# Autodesk Inventor assembly: Lap rap truc Y
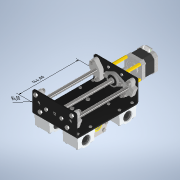
[picture p0: Inventor's stored thumbnail of the model, 180x180]
Saved by Autodesk Inventor 2021 (Build 250183000, 183)
## iProperties
Created: 2021-05-26
Part Number: Lap rap truc Y
Document SubType Name: Assembly
Designer: admin
Author: admin
## Documents named in this file (21)
- C:\Users\79449\Documents\CNC_DISENO_DE MAQUINAS\Piezas-Ensambles_Inventor\Segunda_presentación\Lap rap truc Y.iam
- C:\Users\79449\Documents\CNC_DISENO_DE MAQUINAS\Piezas-Ensambles_Inventor\Segunda_presentación\De  truc Y.ipt
- C:\Users\79449\Documents\CNC_DISENO_DE MAQUINAS\Piezas-Ensambles_Inventor\Segunda_presentación\Kep Truc KLF-08.ipt
- C:\Users\79449\Documents\CNC_DISENO_DE MAQUINAS\Piezas-Ensambles_Inventor\Segunda_presentación\Nema17\Assembly1.iam
- C:\Users\79449\Documents\CNC_DISENO_DE MAQUINAS\Piezas-Ensambles_Inventor\Segunda_presentación\Tru dong 40mm.ipt
- C:\Users\79449\Documents\CNC_DISENO_DE MAQUINAS\Piezas-Ensambles_Inventor\Segunda_presentación\SC12uu\PILLOW 12MM FINAL.iam
- C:\Users\79449\Documents\CNC_DISENO_DE MAQUINAS\Piezas-Ensambles_Inventor\Segunda_presentación\Flexible Coupling 8,8.ipt
- C:\Users\79449\Documents\CNC_DISENO_DE MAQUINAS\Piezas-Ensambles_Inventor\Segunda_presentación\Vitme T8 dai 200mm.ipt
- C:\Users\79449\Documents\CNC_DISENO_DE MAQUINAS\Piezas-Ensambles_Inventor\Segunda_presentación\SHF08.ipt
- C:\Users\79449\Documents\CNC_DISENO_DE MAQUINAS\Piezas-Ensambles_Inventor\Segunda_presentación\EjeBase.ipt
- C:\Users\79449\Documents\CNC_DISENO_DE MAQUINAS\Piezas-Ensambles_Inventor\Segunda_presentación\ball nut housing bracket holder.ipt
- C:\Users\79449\Documents\CNC_DISENO_DE MAQUINAS\Piezas-Ensambles_Inventor\Segunda_presentación\SFU-1605.ipt
- C:\Users\79449\Documents\Inventor\Content Center Files\R2021\es-ES\AS 1110\AS 1110 - M5 x 20.ipt
- C:\Users\79449\Documents\Inventor\Content Center Files\R2021\es-ES\AS 1110\AS 1110 - M2,5 x 6.ipt
- C:\Users\79449\Documents\Inventor\Content Center Files\R2021\es-ES\AS 1110\AS 1110 - M4 x 12.ipt
- C:\Users\79449\Documents\Inventor\Content Center Files\R2021\es-ES\AS 1110\AS 1110 - M3 x 30.ipt
- C:\Users\79449\Documents\Inventor\Content Center Files\R2021\es-ES\AS 1110\AS 1110 - M4 x 8.ipt
- C:\Users\79449\Documents\Inventor\Content Center Files\R2021\es-ES\AS 1110\AS 1110 - M4 x 20.ipt
- C:\Users\79449\Documents\Inventor\Content Center Files\R2021\es-ES\ANSI B18.2.4.2M\ANSI B18.2.4.2M - M5x0,8 - 8.ipt
- C:\Users\79449\Documents\Inventor\Content Center Files\R2021\es-ES\ANSI B18.2.4.2M\ANSI B18.2.4.2M - M4x0,7 - 7.ipt
- C:\Users\79449\Documents\Inventor\Content Center Files\R2021\es-ES\ANSI B18.2.4.2M\ANSI B18.2.4.2M - M3x0,5 - 5,5.ipt
## Components (92 placed, 20 different names)
1. De  truc Y:1 — Mate:4, Mate:5, Mate:6, Mate:13, Mate:15, Mate:16, Mate:21, Mate:22, Mate:23, Mate:24, Mate:25, Mate:26, Mate:27, Mate:28, Mate:37, Mate:38, Mate:39, Mate:48, Mate:53, Mate:54, Mate:57, Mate:58, Mate:59, Mate:60, Mate:63, Mate:64, Mate:65, Ángulo:1, Coincidencia:70, Coincidencia:71, Coincidencia:73, Coincidencia:74, Coincidencia:75, Coincidencia:76, Coincidencia:77, Coincidencia:78, Coincidencia:79, Coincidencia:80, Coincidencia:81, Coincidencia:82, Coincidencia:83, Coincidencia:85, Coincidencia:86, Coincidencia:87, Coincidencia:91, Coincidencia:93, Coincidencia:95, Coincidencia:97, Coincidencia:99, Coincidencia:101, Coincidencia:103, Coincidencia:105, Coincidencia:107, Coincidencia:111, Coincidencia:113, Coincidencia:115, Coincidencia:117, Coincidencia:119, Coincidencia:121, Coincidencia:123, Coincidencia:125, Coincidencia:127, Coincidencia:129, Coincidencia:131, Coincidencia:133, Coincidencia:135, Coincidencia:137, Coincidencia:139, Coincidencia:141, Coincidencia:143, Coincidencia:145, Coincidencia:147, Coincidencia:149, Coincidencia:151, Coincidencia:153, Coincidencia:155, Coincidencia:157, Coincidencia:219, Coincidencia:221, Coincidencia:223, Coincidencia:225
2. Assembly1:1 [sub-assembly] — Coincidencia:69, Ángulo:1
3. Kep Truc KLF-08:2 — Mate:4, Mate:5, Mate:6, Coincidencia:118, Coincidencia:120, Coincidencia:187, Coincidencia:189
4. Kep Truc KLF-08:3 — Mate:13, Mate:15, Mate:16, Mate:19, Coincidencia:122, Coincidencia:124, Coincidencia:191, Coincidencia:193
5. Vitme T8 dai 200mm:1 — Mate:19, Coincidencia:90
6. Tru dong 40mm:1 — Mate:22, Mate:26, Coincidencia:110
7. Tru dong 40mm:2 — Mate:21, Mate:25, Coincidencia:116
8. Tru dong 40mm:3 — Mate:24, Mate:28, Coincidencia:114
9. Tru dong 40mm:4 — Mate:23, Mate:27, Coincidencia:69, Coincidencia:112
10. PILLOW 12MM FINAL:5 [sub-assembly] — Mate:37, Mate:38, Mate:39, Coincidencia:77, Coincidencia:78, Coincidencia:126, Coincidencia:128, Coincidencia:130, Coincidencia:132, Coincidencia:203, Coincidencia:205, Coincidencia:207, Coincidencia:209
11. PILLOW 12MM FINAL:6 [sub-assembly] — Mate:48, Coincidencia:79, Coincidencia:80, Coincidencia:218, Coincidencia:220, Coincidencia:222, Coincidencia:224, Coincidencia:227, Coincidencia:229, Coincidencia:231, Coincidencia:233
12. PILLOW 12MM FINAL:7 [sub-assembly] — Flush:1, Flush:2, Mate:53, Coincidencia:75, Coincidencia:76, Coincidencia:83, Coincidencia:134, Coincidencia:136, Coincidencia:138, Coincidencia:140, Coincidencia:195, Coincidencia:197, Coincidencia:199, Coincidencia:201
13. PILLOW 12MM FINAL:8 [sub-assembly] — Flush:1, Flush:2, Coincidencia:81, Coincidencia:82, Coincidencia:142, Coincidencia:144, Coincidencia:146, Coincidencia:148, Coincidencia:211, Coincidencia:213, Coincidencia:215, Coincidencia:217
14. SHF08:1 — Mate:54, Coincidencia:72, Coincidencia:100, Coincidencia:102, Coincidencia:171, Coincidencia:173
15. SHF08:2 — Mate:60, Coincidencia:74, Coincidencia:92, Coincidencia:94, Coincidencia:183, Coincidencia:185
16. SHF08:3 — Mate:63, Mate:64, Mate:65, Coincidencia:96, Coincidencia:98, Coincidencia:179, Coincidencia:181
17. SHF08:4 — Mate:57, Mate:58, Mate:59, Coincidencia:104, Coincidencia:106, Coincidencia:175, Coincidencia:177
18. EjeBase:1 — Coincidencia:70, Coincidencia:71
19. EjeBase:2 — Coincidencia:72, Coincidencia:73
20. ball nut housing bracket holder:1 — Coincidencia:85, Coincidencia:86, Coincidencia:87, Coincidencia:88, Ángulo:2, Coincidencia:89, Coincidencia:150, Coincidencia:152, Coincidencia:154, Coincidencia:156, Coincidencia:158, Coincidencia:160, Coincidencia:162, Coincidencia:164, Coincidencia:166, Coincidencia:168
21. SFU-1605:1 — Coincidencia:88, Ángulo:2, Coincidencia:89, Coincidencia:159, Coincidencia:161, Coincidencia:163, Coincidencia:165, Coincidencia:167, Coincidencia:169
22. Flexible Coupling 8,8:1 — Coincidencia:90, Coincidencia:91
23. AS 1110 - Métrico M5 x 20:1 — Coincidencia:92, Coincidencia:93, Coincidencia:182
24. AS 1110 - Métrico M5 x 20:2 — Coincidencia:94, Coincidencia:95, Coincidencia:184
25. AS 1110 - Métrico M5 x 20:3 — Coincidencia:96, Coincidencia:97, Coincidencia:178
26. AS 1110 - Métrico M5 x 20:4 — Coincidencia:98, Coincidencia:99, Coincidencia:180
27. AS 1110 - Métrico M5 x 20:5 — Coincidencia:100, Coincidencia:101, Coincidencia:170
28. AS 1110 - Métrico M5 x 20:6 — Coincidencia:102, Coincidencia:103, Coincidencia:172
29. AS 1110 - Métrico M5 x 20:7 — Coincidencia:104, Coincidencia:105, Coincidencia:174
30. AS 1110 - Métrico M5 x 20:8 — Coincidencia:106, Coincidencia:107, Coincidencia:176
31. AS 1110 - Métrico M2,5 x 6:2 — Coincidencia:110, Coincidencia:111
32. AS 1110 - Métrico M2,5 x 6:3 — Coincidencia:112, Coincidencia:113
33. AS 1110 - Métrico M2,5 x 6:4 — Coincidencia:114, Coincidencia:115
34. AS 1110 - Métrico M2,5 x 6:5 — Coincidencia:116, Coincidencia:117
35. AS 1110 - Métrico M4 x 12:1 — Coincidencia:118, Coincidencia:119, Coincidencia:188
36. AS 1110 - Métrico M4 x 12:2 — Coincidencia:120, Coincidencia:121, Coincidencia:186
37. AS 1110 - Métrico M4 x 12:3 — Coincidencia:122, Coincidencia:123, Coincidencia:192
38. AS 1110 - Métrico M4 x 12:4 — Coincidencia:124, Coincidencia:125, Coincidencia:190
39. AS 1110 - Métrico M3 x 30:1 — Coincidencia:126, Coincidencia:127, Coincidencia:206
40. AS 1110 - Métrico M3 x 30:2 — Coincidencia:128, Coincidencia:129, Coincidencia:208
41. AS 1110 - Métrico M3 x 30:3 — Coincidencia:130, Coincidencia:131, Coincidencia:204
42. AS 1110 - Métrico M3 x 30:4 — Coincidencia:132, Coincidencia:133, Coincidencia:202
43. AS 1110 - Métrico M3 x 30:5 — Coincidencia:134, Coincidencia:135, Coincidencia:194
44. AS 1110 - Métrico M3 x 30:6 — Coincidencia:136, Coincidencia:137, Coincidencia:196
45. AS 1110 - Métrico M3 x 30:7 — Coincidencia:138, Coincidencia:139, Coincidencia:200
46. AS 1110 - Métrico M3 x 30:8 — Coincidencia:140, Coincidencia:141, Coincidencia:198
47. AS 1110 - Métrico M3 x 30:9 — Coincidencia:142, Coincidencia:143, Coincidencia:216
48. AS 1110 - Métrico M3 x 30:10 — Coincidencia:144, Coincidencia:145, Coincidencia:210
49. AS 1110 - Métrico M3 x 30:11 — Coincidencia:146, Coincidencia:147, Coincidencia:214
50. AS 1110 - Métrico M3 x 30:12 — Coincidencia:148, Coincidencia:149, Coincidencia:212
51. AS 1110 - Métrico M4 x 8:1 — Coincidencia:150, Coincidencia:151
52. AS 1110 - Métrico M4 x 8:2 — Coincidencia:152, Coincidencia:153
53. AS 1110 - Métrico M4 x 8:3 — Coincidencia:154, Coincidencia:155
54. AS 1110 - Métrico M4 x 8:4 — Coincidencia:156, Coincidencia:157
55. AS 1110 - Métrico M4 x 20:1 — Coincidencia:158, Coincidencia:159
56. AS 1110 - Métrico M4 x 20:2 — Coincidencia:160, Coincidencia:161
57. AS 1110 - Métrico M4 x 20:3 — Coincidencia:162, Coincidencia:163
58. AS 1110 - Métrico M4 x 20:4 — Coincidencia:164, Coincidencia:165
59. AS 1110 - Métrico M4 x 20:5 — Coincidencia:166, Coincidencia:167
60. AS 1110 - Métrico M4 x 20:6 — Coincidencia:168, Coincidencia:169
61. ANSI B18.2.4.2M M5x0,8:1 — Coincidencia:170, Coincidencia:171
62. ANSI B18.2.4.2M M5x0,8:2 — Coincidencia:172, Coincidencia:173
63. ANSI B18.2.4.2M M5x0,8:3 — Coincidencia:174, Coincidencia:175
64. ANSI B18.2.4.2M M5x0,8:4 — Coincidencia:176, Coincidencia:177
65. ANSI B18.2.4.2M M5x0,8:5 — Coincidencia:178, Coincidencia:179
66. ANSI B18.2.4.2M M5x0,8:6 — Coincidencia:180, Coincidencia:181
67. ANSI B18.2.4.2M M5x0,8:7 — Coincidencia:182, Coincidencia:183
68. ANSI B18.2.4.2M M5x0,8:8 — Coincidencia:184, Coincidencia:185
69. ANSI B18.2.4.2M M4x0,7:1 — Coincidencia:186, Coincidencia:187
70. ANSI B18.2.4.2M M4x0,7:2 — Coincidencia:188, Coincidencia:189
71. ANSI B18.2.4.2M M4x0,7:3 — Coincidencia:190, Coincidencia:191
72. ANSI B18.2.4.2M M4x0,7:4 — Coincidencia:192, Coincidencia:193
73. ANSI B18.2.4.2M M3x0,5:1 — Coincidencia:194, Coincidencia:195
74. ANSI B18.2.4.2M M3x0,5:2 — Coincidencia:196, Coincidencia:197
75. ANSI B18.2.4.2M M3x0,5:3 — Coincidencia:198, Coincidencia:199
76. ANSI B18.2.4.2M M3x0,5:4 — Coincidencia:200, Coincidencia:201
77. ANSI B18.2.4.2M M3x0,5:5 — Coincidencia:202, Coincidencia:203
78. ANSI B18.2.4.2M M3x0,5:6 — Coincidencia:204, Coincidencia:205
79. ANSI B18.2.4.2M M3x0,5:7 — Coincidencia:206, Coincidencia:207
80. ANSI B18.2.4.2M M3x0,5:8 — Coincidencia:208, Coincidencia:209
81. ANSI B18.2.4.2M M3x0,5:9 — Coincidencia:210, Coincidencia:211
82. ANSI B18.2.4.2M M3x0,5:10 — Coincidencia:212, Coincidencia:213
83. ANSI B18.2.4.2M M3x0,5:11 — Coincidencia:214, Coincidencia:215
84. ANSI B18.2.4.2M M3x0,5:12 — Coincidencia:216, Coincidencia:217
85. AS 1110 - Métrico M3 x 30:13 — Coincidencia:218, Coincidencia:219, Coincidencia:232
86. AS 1110 - Métrico M3 x 30:14 — Coincidencia:220, Coincidencia:221, Coincidencia:230
87. AS 1110 - Métrico M3 x 30:15 — Coincidencia:222, Coincidencia:223, Coincidencia:226
88. AS 1110 - Métrico M3 x 30:16 — Coincidencia:224, Coincidencia:225, Coincidencia:228
89. ANSI B18.2.4.2M M3x0,5:13 — Coincidencia:226, Coincidencia:227
90. ANSI B18.2.4.2M M3x0,5:14 — Coincidencia:228, Coincidencia:229
91. ANSI B18.2.4.2M M3x0,5:15 — Coincidencia:230, Coincidencia:231
92. ANSI B18.2.4.2M M3x0,5:16 — Coincidencia:232, Coincidencia:233
## Relationships (194: Mate 190, Flush 2, Angle 2)
- Mate:4: De  truc Y:1 ↔ Kep Truc KLF-08:2
- Mate:5: De  truc Y:1 ↔ Kep Truc KLF-08:2
- Mate:6: De  truc Y:1 ↔ Kep Truc KLF-08:2
- Mate:13: De  truc Y:1 ↔ Kep Truc KLF-08:3
- Mate:15: De  truc Y:1 ↔ Kep Truc KLF-08:3
- Mate:16: De  truc Y:1 ↔ Kep Truc KLF-08:3
- Mate:19: Kep Truc KLF-08:3 ↔ Vitme T8 dai 200mm:1
- Mate:21: De  truc Y:1 ↔ Tru dong 40mm:2
- Mate:22: De  truc Y:1 ↔ Tru dong 40mm:1
- Mate:23: De  truc Y:1 ↔ Tru dong 40mm:4
- Mate:24: De  truc Y:1 ↔ Tru dong 40mm:3
- Mate:25: De  truc Y:1 ↔ Tru dong 40mm:2
- Mate:26: De  truc Y:1 ↔ Tru dong 40mm:1
- Mate:27: De  truc Y:1 ↔ Tru dong 40mm:4
- Mate:28: De  truc Y:1 ↔ Tru dong 40mm:3
- Mate:37: De  truc Y:1 ↔ PILLOW 12MM FINAL:5
- Mate:38: De  truc Y:1 ↔ PILLOW 12MM FINAL:5
- Mate:39: De  truc Y:1 ↔ PILLOW 12MM FINAL:5
- Mate:48: De  truc Y:1 ↔ PILLOW 12MM FINAL:6
- Flush:1: PILLOW 12MM FINAL:7 ↔ PILLOW 12MM FINAL:8
- Flush:2: PILLOW 12MM FINAL:7 ↔ PILLOW 12MM FINAL:8
- Mate:53: De  truc Y:1 ↔ PILLOW 12MM FINAL:7
- Mate:54: De  truc Y:1 ↔ SHF08:1
- Mate:57: De  truc Y:1 ↔ SHF08:4
- Mate:58: De  truc Y:1 ↔ SHF08:4
- Mate:59: De  truc Y:1 ↔ SHF08:4
- Mate:60: De  truc Y:1 ↔ SHF08:2
- Mate:63: De  truc Y:1 ↔ SHF08:3
- Mate:64: De  truc Y:1 ↔ SHF08:3
- Mate:65: De  truc Y:1 ↔ SHF08:3
- Coincidencia:69 [Mate]: Assembly1:1 ↔ Tru dong 40mm:4
- Ángulo:1 [Angle] (0 deg): De  truc Y:1 ↔ Assembly1:1
- Coincidencia:70 [Mate]: De  truc Y:1 ↔ EjeBase:1
- Coincidencia:71 [Mate]: De  truc Y:1 ↔ EjeBase:1
- Coincidencia:72 [Mate]: SHF08:1 ↔ EjeBase:2
- Coincidencia:73 [Mate]: De  truc Y:1 ↔ EjeBase:2
- Coincidencia:74 [Mate]: De  truc Y:1 ↔ SHF08:2
- Coincidencia:75 [Mate]: De  truc Y:1 ↔ PILLOW 12MM FINAL:7
- Coincidencia:76 [Mate]: De  truc Y:1 ↔ PILLOW 12MM FINAL:7
- Coincidencia:77 [Mate]: De  truc Y:1 ↔ PILLOW 12MM FINAL:5
- Coincidencia:78 [Mate]: De  truc Y:1 ↔ PILLOW 12MM FINAL:5
- Coincidencia:79 [Mate]: De  truc Y:1 ↔ PILLOW 12MM FINAL:6
- Coincidencia:80 [Mate]: De  truc Y:1 ↔ PILLOW 12MM FINAL:6
- Coincidencia:81 [Mate]: De  truc Y:1 ↔ PILLOW 12MM FINAL:8
- Coincidencia:82 [Mate]: De  truc Y:1 ↔ PILLOW 12MM FINAL:8
- Coincidencia:83 [Mate]: De  truc Y:1 ↔ PILLOW 12MM FINAL:7
- Coincidencia:85 [Mate]: De  truc Y:1 ↔ ball nut housing bracket holder:1
- Coincidencia:86 [Mate]: De  truc Y:1 ↔ ball nut housing bracket holder:1
- Coincidencia:87 [Mate]: De  truc Y:1 ↔ ball nut housing bracket holder:1
- Coincidencia:88 [Mate]: ball nut housing bracket holder:1 ↔ SFU-1605:1
- Ángulo:2 [Angle] (0 deg): ball nut housing bracket holder:1 ↔ SFU-1605:1
- Coincidencia:89 [Mate]: ball nut housing bracket holder:1 ↔ SFU-1605:1
- Coincidencia:90 [Mate]: Vitme T8 dai 200mm:1 ↔ Flexible Coupling 8,8:1
- Coincidencia:91 [Mate]: De  truc Y:1 ↔ Flexible Coupling 8,8:1
- Coincidencia:92 [Mate]: SHF08:2 ↔ AS 1110 - Métrico M5 x 20:1
- Coincidencia:93 [Mate]: De  truc Y:1 ↔ AS 1110 - Métrico M5 x 20:1
- Coincidencia:94 [Mate]: SHF08:2 ↔ AS 1110 - Métrico M5 x 20:2
- Coincidencia:95 [Mate]: De  truc Y:1 ↔ AS 1110 - Métrico M5 x 20:2
- Coincidencia:96 [Mate]: SHF08:3 ↔ AS 1110 - Métrico M5 x 20:3
- Coincidencia:97 [Mate]: De  truc Y:1 ↔ AS 1110 - Métrico M5 x 20:3
- Coincidencia:98 [Mate]: SHF08:3 ↔ AS 1110 - Métrico M5 x 20:4
- Coincidencia:99 [Mate]: De  truc Y:1 ↔ AS 1110 - Métrico M5 x 20:4
- Coincidencia:100 [Mate]: SHF08:1 ↔ AS 1110 - Métrico M5 x 20:5
- Coincidencia:101 [Mate]: De  truc Y:1 ↔ AS 1110 - Métrico M5 x 20:5
- Coincidencia:102 [Mate]: SHF08:1 ↔ AS 1110 - Métrico M5 x 20:6
- Coincidencia:103 [Mate]: De  truc Y:1 ↔ AS 1110 - Métrico M5 x 20:6
- Coincidencia:104 [Mate]: SHF08:4 ↔ AS 1110 - Métrico M5 x 20:7
- Coincidencia:105 [Mate]: De  truc Y:1 ↔ AS 1110 - Métrico M5 x 20:7
- Coincidencia:106 [Mate]: SHF08:4 ↔ AS 1110 - Métrico M5 x 20:8
- Coincidencia:107 [Mate]: De  truc Y:1 ↔ AS 1110 - Métrico M5 x 20:8
- Coincidencia:110 [Mate]: Tru dong 40mm:1 ↔ AS 1110 - Métrico M2,5 x 6:2
- Coincidencia:111 [Mate]: De  truc Y:1 ↔ AS 1110 - Métrico M2,5 x 6:2
- Coincidencia:112 [Mate]: Tru dong 40mm:4 ↔ AS 1110 - Métrico M2,5 x 6:3
- Coincidencia:113 [Mate]: De  truc Y:1 ↔ AS 1110 - Métrico M2,5 x 6:3
- Coincidencia:114 [Mate]: Tru dong 40mm:3 ↔ AS 1110 - Métrico M2,5 x 6:4
- Coincidencia:115 [Mate]: De  truc Y:1 ↔ AS 1110 - Métrico M2,5 x 6:4
- Coincidencia:116 [Mate]: Tru dong 40mm:2 ↔ AS 1110 - Métrico M2,5 x 6:5
- Coincidencia:117 [Mate]: De  truc Y:1 ↔ AS 1110 - Métrico M2,5 x 6:5
- Coincidencia:118 [Mate]: Kep Truc KLF-08:2 ↔ AS 1110 - Métrico M4 x 12:1
- Coincidencia:119 [Mate]: De  truc Y:1 ↔ AS 1110 - Métrico M4 x 12:1
- Coincidencia:120 [Mate]: Kep Truc KLF-08:2 ↔ AS 1110 - Métrico M4 x 12:2
- Coincidencia:121 [Mate]: De  truc Y:1 ↔ AS 1110 - Métrico M4 x 12:2
- Coincidencia:122 [Mate]: Kep Truc KLF-08:3 ↔ AS 1110 - Métrico M4 x 12:3
- Coincidencia:123 [Mate]: De  truc Y:1 ↔ AS 1110 - Métrico M4 x 12:3
- Coincidencia:124 [Mate]: Kep Truc KLF-08:3 ↔ AS 1110 - Métrico M4 x 12:4
- Coincidencia:125 [Mate]: De  truc Y:1 ↔ AS 1110 - Métrico M4 x 12:4
- Coincidencia:126 [Mate]: PILLOW 12MM FINAL:5 ↔ AS 1110 - Métrico M3 x 30:1
- Coincidencia:127 [Mate]: De  truc Y:1 ↔ AS 1110 - Métrico M3 x 30:1
- Coincidencia:128 [Mate]: PILLOW 12MM FINAL:5 ↔ AS 1110 - Métrico M3 x 30:2
- Coincidencia:129 [Mate]: De  truc Y:1 ↔ AS 1110 - Métrico M3 x 30:2
- Coincidencia:130 [Mate]: PILLOW 12MM FINAL:5 ↔ AS 1110 - Métrico M3 x 30:3
- Coincidencia:131 [Mate]: De  truc Y:1 ↔ AS 1110 - Métrico M3 x 30:3
- Coincidencia:132 [Mate]: PILLOW 12MM FINAL:5 ↔ AS 1110 - Métrico M3 x 30:4
- Coincidencia:133 [Mate]: De  truc Y:1 ↔ AS 1110 - Métrico M3 x 30:4
- Coincidencia:134 [Mate]: PILLOW 12MM FINAL:7 ↔ AS 1110 - Métrico M3 x 30:5
- Coincidencia:135 [Mate]: De  truc Y:1 ↔ AS 1110 - Métrico M3 x 30:5
- Coincidencia:136 [Mate]: PILLOW 12MM FINAL:7 ↔ AS 1110 - Métrico M3 x 30:6
- Coincidencia:137 [Mate]: De  truc Y:1 ↔ AS 1110 - Métrico M3 x 30:6
- Coincidencia:138 [Mate]: PILLOW 12MM FINAL:7 ↔ AS 1110 - Métrico M3 x 30:7
- Coincidencia:139 [Mate]: De  truc Y:1 ↔ AS 1110 - Métrico M3 x 30:7
- Coincidencia:140 [Mate]: PILLOW 12MM FINAL:7 ↔ AS 1110 - Métrico M3 x 30:8
- Coincidencia:141 [Mate]: De  truc Y:1 ↔ AS 1110 - Métrico M3 x 30:8
- Coincidencia:142 [Mate]: PILLOW 12MM FINAL:8 ↔ AS 1110 - Métrico M3 x 30:9
- Coincidencia:143 [Mate]: De  truc Y:1 ↔ AS 1110 - Métrico M3 x 30:9
- Coincidencia:144 [Mate]: PILLOW 12MM FINAL:8 ↔ AS 1110 - Métrico M3 x 30:10
- Coincidencia:145 [Mate]: De  truc Y:1 ↔ AS 1110 - Métrico M3 x 30:10
- Coincidencia:146 [Mate]: PILLOW 12MM FINAL:8 ↔ AS 1110 - Métrico M3 x 30:11
- Coincidencia:147 [Mate]: De  truc Y:1 ↔ AS 1110 - Métrico M3 x 30:11
- Coincidencia:148 [Mate]: PILLOW 12MM FINAL:8 ↔ AS 1110 - Métrico M3 x 30:12
- Coincidencia:149 [Mate]: De  truc Y:1 ↔ AS 1110 - Métrico M3 x 30:12
- Coincidencia:150 [Mate]: ball nut housing bracket holder:1 ↔ AS 1110 - Métrico M4 x 8:1
- Coincidencia:151 [Mate]: De  truc Y:1 ↔ AS 1110 - Métrico M4 x 8:1
- Coincidencia:152 [Mate]: ball nut housing bracket holder:1 ↔ AS 1110 - Métrico M4 x 8:2
- Coincidencia:153 [Mate]: De  truc Y:1 ↔ AS 1110 - Métrico M4 x 8:2
- Coincidencia:154 [Mate]: ball nut housing bracket holder:1 ↔ AS 1110 - Métrico M4 x 8:3
- Coincidencia:155 [Mate]: De  truc Y:1 ↔ AS 1110 - Métrico M4 x 8:3
- Coincidencia:156 [Mate]: ball nut housing bracket holder:1 ↔ AS 1110 - Métrico M4 x 8:4
- Coincidencia:157 [Mate]: De  truc Y:1 ↔ AS 1110 - Métrico M4 x 8:4
- Coincidencia:158 [Mate]: ball nut housing bracket holder:1 ↔ AS 1110 - Métrico M4 x 20:1
- Coincidencia:159 [Mate]: SFU-1605:1 ↔ AS 1110 - Métrico M4 x 20:1
- Coincidencia:160 [Mate]: ball nut housing bracket holder:1 ↔ AS 1110 - Métrico M4 x 20:2
- Coincidencia:161 [Mate]: SFU-1605:1 ↔ AS 1110 - Métrico M4 x 20:2
- Coincidencia:162 [Mate]: ball nut housing bracket holder:1 ↔ AS 1110 - Métrico M4 x 20:3
- Coincidencia:163 [Mate]: SFU-1605:1 ↔ AS 1110 - Métrico M4 x 20:3
- Coincidencia:164 [Mate]: ball nut housing bracket holder:1 ↔ AS 1110 - Métrico M4 x 20:4
- Coincidencia:165 [Mate]: SFU-1605:1 ↔ AS 1110 - Métrico M4 x 20:4
- Coincidencia:166 [Mate]: ball nut housing bracket holder:1 ↔ AS 1110 - Métrico M4 x 20:5
- Coincidencia:167 [Mate]: SFU-1605:1 ↔ AS 1110 - Métrico M4 x 20:5
- Coincidencia:168 [Mate]: ball nut housing bracket holder:1 ↔ AS 1110 - Métrico M4 x 20:6
- Coincidencia:169 [Mate]: SFU-1605:1 ↔ AS 1110 - Métrico M4 x 20:6
- Coincidencia:170 [Mate]: AS 1110 - Métrico M5 x 20:5 ↔ ANSI B18.2.4.2M M5x0,8:1
- Coincidencia:171 [Mate]: SHF08:1 ↔ ANSI B18.2.4.2M M5x0,8:1
- Coincidencia:172 [Mate]: AS 1110 - Métrico M5 x 20:6 ↔ ANSI B18.2.4.2M M5x0,8:2
- Coincidencia:173 [Mate]: SHF08:1 ↔ ANSI B18.2.4.2M M5x0,8:2
- Coincidencia:174 [Mate]: AS 1110 - Métrico M5 x 20:7 ↔ ANSI B18.2.4.2M M5x0,8:3
- Coincidencia:175 [Mate]: SHF08:4 ↔ ANSI B18.2.4.2M M5x0,8:3
- Coincidencia:176 [Mate]: AS 1110 - Métrico M5 x 20:8 ↔ ANSI B18.2.4.2M M5x0,8:4
- Coincidencia:177 [Mate]: SHF08:4 ↔ ANSI B18.2.4.2M M5x0,8:4
- Coincidencia:178 [Mate]: AS 1110 - Métrico M5 x 20:3 ↔ ANSI B18.2.4.2M M5x0,8:5
- Coincidencia:179 [Mate]: SHF08:3 ↔ ANSI B18.2.4.2M M5x0,8:5
- Coincidencia:180 [Mate]: AS 1110 - Métrico M5 x 20:4 ↔ ANSI B18.2.4.2M M5x0,8:6
- Coincidencia:181 [Mate]: SHF08:3 ↔ ANSI B18.2.4.2M M5x0,8:6
- Coincidencia:182 [Mate]: AS 1110 - Métrico M5 x 20:1 ↔ ANSI B18.2.4.2M M5x0,8:7
- Coincidencia:183 [Mate]: SHF08:2 ↔ ANSI B18.2.4.2M M5x0,8:7
- Coincidencia:184 [Mate]: AS 1110 - Métrico M5 x 20:2 ↔ ANSI B18.2.4.2M M5x0,8:8
- Coincidencia:185 [Mate]: SHF08:2 ↔ ANSI B18.2.4.2M M5x0,8:8
- Coincidencia:186 [Mate]: AS 1110 - Métrico M4 x 12:2 ↔ ANSI B18.2.4.2M M4x0,7:1
- Coincidencia:187 [Mate]: Kep Truc KLF-08:2 ↔ ANSI B18.2.4.2M M4x0,7:1
- Coincidencia:188 [Mate]: AS 1110 - Métrico M4 x 12:1 ↔ ANSI B18.2.4.2M M4x0,7:2
- Coincidencia:189 [Mate]: Kep Truc KLF-08:2 ↔ ANSI B18.2.4.2M M4x0,7:2
- Coincidencia:190 [Mate]: AS 1110 - Métrico M4 x 12:4 ↔ ANSI B18.2.4.2M M4x0,7:3
- Coincidencia:191 [Mate]: Kep Truc KLF-08:3 ↔ ANSI B18.2.4.2M M4x0,7:3
- Coincidencia:192 [Mate]: AS 1110 - Métrico M4 x 12:3 ↔ ANSI B18.2.4.2M M4x0,7:4
- Coincidencia:193 [Mate]: Kep Truc KLF-08:3 ↔ ANSI B18.2.4.2M M4x0,7:4
- Coincidencia:194 [Mate]: AS 1110 - Métrico M3 x 30:5 ↔ ANSI B18.2.4.2M M3x0,5:1
- Coincidencia:195 [Mate]: PILLOW 12MM FINAL:7 ↔ ANSI B18.2.4.2M M3x0,5:1
- Coincidencia:196 [Mate]: AS 1110 - Métrico M3 x 30:6 ↔ ANSI B18.2.4.2M M3x0,5:2
- Coincidencia:197 [Mate]: PILLOW 12MM FINAL:7 ↔ ANSI B18.2.4.2M M3x0,5:2
- Coincidencia:198 [Mate]: AS 1110 - Métrico M3 x 30:8 ↔ ANSI B18.2.4.2M M3x0,5:3
- Coincidencia:199 [Mate]: PILLOW 12MM FINAL:7 ↔ ANSI B18.2.4.2M M3x0,5:3
- Coincidencia:200 [Mate]: AS 1110 - Métrico M3 x 30:7 ↔ ANSI B18.2.4.2M M3x0,5:4
- Coincidencia:201 [Mate]: PILLOW 12MM FINAL:7 ↔ ANSI B18.2.4.2M M3x0,5:4
- Coincidencia:202 [Mate]: AS 1110 - Métrico M3 x 30:4 ↔ ANSI B18.2.4.2M M3x0,5:5
- Coincidencia:203 [Mate]: PILLOW 12MM FINAL:5 ↔ ANSI B18.2.4.2M M3x0,5:5
- Coincidencia:204 [Mate]: AS 1110 - Métrico M3 x 30:3 ↔ ANSI B18.2.4.2M M3x0,5:6
- Coincidencia:205 [Mate]: PILLOW 12MM FINAL:5 ↔ ANSI B18.2.4.2M M3x0,5:6
- Coincidencia:206 [Mate]: AS 1110 - Métrico M3 x 30:1 ↔ ANSI B18.2.4.2M M3x0,5:7
- Coincidencia:207 [Mate]: PILLOW 12MM FINAL:5 ↔ ANSI B18.2.4.2M M3x0,5:7
- Coincidencia:208 [Mate]: AS 1110 - Métrico M3 x 30:2 ↔ ANSI B18.2.4.2M M3x0,5:8
- Coincidencia:209 [Mate]: PILLOW 12MM FINAL:5 ↔ ANSI B18.2.4.2M M3x0,5:8
- Coincidencia:210 [Mate]: AS 1110 - Métrico M3 x 30:10 ↔ ANSI B18.2.4.2M M3x0,5:9
- Coincidencia:211 [Mate]: PILLOW 12MM FINAL:8 ↔ ANSI B18.2.4.2M M3x0,5:9
- Coincidencia:212 [Mate]: AS 1110 - Métrico M3 x 30:12 ↔ ANSI B18.2.4.2M M3x0,5:10
- Coincidencia:213 [Mate]: PILLOW 12MM FINAL:8 ↔ ANSI B18.2.4.2M M3x0,5:10
- Coincidencia:214 [Mate]: AS 1110 - Métrico M3 x 30:11 ↔ ANSI B18.2.4.2M M3x0,5:11
- Coincidencia:215 [Mate]: PILLOW 12MM FINAL:8 ↔ ANSI B18.2.4.2M M3x0,5:11
- Coincidencia:216 [Mate]: AS 1110 - Métrico M3 x 30:9 ↔ ANSI B18.2.4.2M M3x0,5:12
- Coincidencia:217 [Mate]: PILLOW 12MM FINAL:8 ↔ ANSI B18.2.4.2M M3x0,5:12
- Coincidencia:218 [Mate]: PILLOW 12MM FINAL:6 ↔ AS 1110 - Métrico M3 x 30:13
- Coincidencia:219 [Mate]: De  truc Y:1 ↔ AS 1110 - Métrico M3 x 30:13
- Coincidencia:220 [Mate]: PILLOW 12MM FINAL:6 ↔ AS 1110 - Métrico M3 x 30:14
- Coincidencia:221 [Mate]: De  truc Y:1 ↔ AS 1110 - Métrico M3 x 30:14
- Coincidencia:222 [Mate]: PILLOW 12MM FINAL:6 ↔ AS 1110 - Métrico M3 x 30:15
- Coincidencia:223 [Mate]: De  truc Y:1 ↔ AS 1110 - Métrico M3 x 30:15
- Coincidencia:224 [Mate]: PILLOW 12MM FINAL:6 ↔ AS 1110 - Métrico M3 x 30:16
- Coincidencia:225 [Mate]: De  truc Y:1 ↔ AS 1110 - Métrico M3 x 30:16
- Coincidencia:226 [Mate]: AS 1110 - Métrico M3 x 30:15 ↔ ANSI B18.2.4.2M M3x0,5:13
- Coincidencia:227 [Mate]: PILLOW 12MM FINAL:6 ↔ ANSI B18.2.4.2M M3x0,5:13
- Coincidencia:228 [Mate]: AS 1110 - Métrico M3 x 30:16 ↔ ANSI B18.2.4.2M M3x0,5:14
- Coincidencia:229 [Mate]: PILLOW 12MM FINAL:6 ↔ ANSI B18.2.4.2M M3x0,5:14
- Coincidencia:230 [Mate]: AS 1110 - Métrico M3 x 30:14 ↔ ANSI B18.2.4.2M M3x0,5:15
- Coincidencia:231 [Mate]: PILLOW 12MM FINAL:6 ↔ ANSI B18.2.4.2M M3x0,5:15
- Coincidencia:232 [Mate]: AS 1110 - Métrico M3 x 30:13 ↔ ANSI B18.2.4.2M M3x0,5:16
- Coincidencia:233 [Mate]: PILLOW 12MM FINAL:6 ↔ ANSI B18.2.4.2M M3x0,5:16
